# Autodesk Inventor assembly: TestSetup
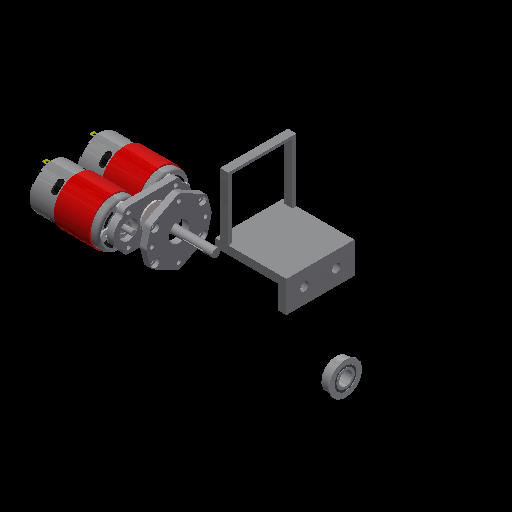
[picture p0: Inventor's stored thumbnail of the model, 512x512]
Saved by Autodesk Inventor 2023 (Build 270158030, 158C)
## iProperties
Created: 2021-12-06
Part Number: TestSetup
Document SubType Name: Assembly
Designer: kumpu
Author: kumpu
## Documents named in this file (9)
- C:\Users\kumpu\Documents\SBU\CAD\SBRT\Robocup Rescue\Drive\v1\DeCIMate.iam
- C:\Users\kumpu\Documents\SBU\CAD\SBRT\Robocup Rescue\Drive\TestSetup1\am-4465 1-2 in ID 1 1-8 in OD Sealed Flanged Bearing FR82RS.ipt
- C:\Users\kumpu\Documents\SBU\CAD\SBRT\Robocup Rescue\Drive\TestSetup1\am-3692 DeCIMate Output Plate.ipt
- C:\Users\kumpu\Documents\SBU\CAD\SBRT\Robocup Rescue\Drive\TestSetup1\am-3693 DeCIMate Motor Plate.ipt
- C:\Users\kumpu\Documents\SBU\CAD\SBRT\Robocup Rescue\Drive\TestSetup1\am-3650 775 Motor Vent Plate.ipt
- C:\Users\kumpu\Documents\SBU\CAD\SBRT\Robocup Rescue\Drive\TestSetup1\am-3775a AndyMark RedLine Motor.ipt
- C:\Users\kumpu\Documents\SBU\CAD\SBRT\Robocup Rescue\Drive\TestSetup1\am-0028 00.375'' id Flanged, Shielded Ball Bearing (FR6ZZ).ipt
- C:\Users\kumpu\Documents\SBU\CAD\SBRT\Robocup Rescue\Drive\TestSetup1\am-3695 DeCIMate Output Shaft.ipt
- C:\Users\kumpu\Documents\SBU\CAD\SBRT\Robocup Rescue\Drive\TestSetup1\B2_RCR_v1.ipt
## Components (10 placed, 8 different names)
1. am-3692 DeCIMate Output Plate:1 — Insert:5, Insert:6, Flush:1, Mate:2
2. am-3693 DeCIMate Motor Plate:1 — Insert:5, Insert:6, Insert:7, Insert:8, Insert:9, Insert:10, Insert:15
3. am-3650 775 Motor Vent Plate:1 — Insert:8, Insert:9, Insert:11, Insert:12
4. am-3775a AndyMark RedLine Motor:1 — Insert:13, Insert:14
5. am-3650 775 Motor Vent Plate:2 — Insert:7, Insert:10, Insert:13, Insert:14
6. am-3775a AndyMark RedLine Motor:2 — Insert:11, Insert:12
7. am-0028 00.375'' id Flanged, Shielded Ball Bearing (FR6ZZ):1 — Insert:15, Insert:16
8. am-3695 DeCIMate Output Shaft:1 — Insert:16, Mate:1
9. am-4465 1-2 in ID 1 1-8 in OD Sealed Flanged Bearing FR82RS:2
10. B2_RCR_v1:1
## Relationships (15: Insert 12, Mate 2, Flush 1)
- Insert:5 (19.05 mm): am-3692 DeCIMate Output Plate:1 ↔ am-3693 DeCIMate Motor Plate:1
- Insert:6 (19.05 mm): am-3692 DeCIMate Output Plate:1 ↔ am-3693 DeCIMate Motor Plate:1
- Insert:7: am-3693 DeCIMate Motor Plate:1 ↔ am-3650 775 Motor Vent Plate:2
- Insert:8: am-3693 DeCIMate Motor Plate:1 ↔ am-3650 775 Motor Vent Plate:1
- Insert:9: am-3693 DeCIMate Motor Plate:1 ↔ am-3650 775 Motor Vent Plate:1
- Insert:10: am-3693 DeCIMate Motor Plate:1 ↔ am-3650 775 Motor Vent Plate:2
- Insert:11: am-3650 775 Motor Vent Plate:1 ↔ am-3775a AndyMark RedLine Motor:2
- Insert:12: am-3650 775 Motor Vent Plate:1 ↔ am-3775a AndyMark RedLine Motor:2
- Insert:13: am-3775a AndyMark RedLine Motor:1 ↔ am-3650 775 Motor Vent Plate:2
- Insert:14: am-3775a AndyMark RedLine Motor:1 ↔ am-3650 775 Motor Vent Plate:2
- Insert:15: am-3693 DeCIMate Motor Plate:1 ↔ am-0028 00.375'' id Flanged, Shielded Ball Bearing (FR6ZZ):1
- Insert:16: am-0028 00.375'' id Flanged, Shielded Ball Bearing (FR6ZZ):1 ↔ am-3695 DeCIMate Output Shaft:1
- Mate:1: am-3695 DeCIMate Output Shaft:1
- Flush:1: am-3692 DeCIMate Output Plate:1
- Mate:2: am-3692 DeCIMate Output Plate:1
